# Autodesk Inventor assembly: A-01-0
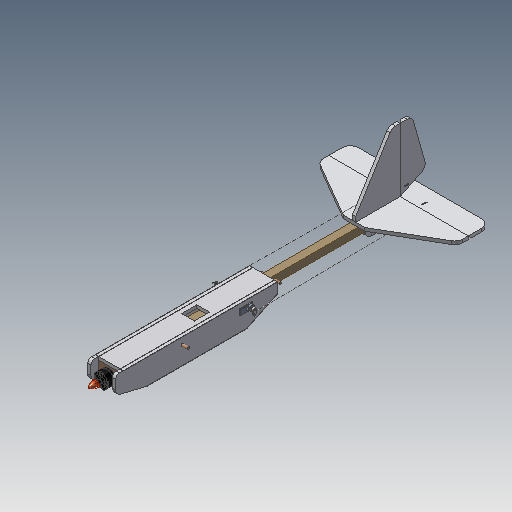
[picture p0: Inventor's stored thumbnail of the model, 512x512]
Saved by Autodesk Inventor 2019 (Build 230136000, 136)
## iProperties
Created: 2022-04-10
Part Number: A-01-0
Document SubType Name: Assembly
Designer: solyo
Mass: 81.7196 g
Surface Area: 1876.72 cm^2
Volume: 370.282 cm^3
Density: 0.220695 g/cm^3
Author: solyo
## Documents named in this file (22)
- D:\Modelling\RC\RC Trainer V1\ASSEMBLY\A-01-0-FUSELAGE\A-01-0.iam
- D:\Modelling\RC\RC Trainer V1\Parts\PW-00-0-TAILBOOM\PW-00-0-0.ipt
- D:\Modelling\RC\RC Trainer V1\Parts\PW-01-0-FIREWALL\PW-01-0-0.ipt
- D:\Modelling\RC\RC Trainer V1\PARTS\PW-02-0-PIN\PW-02-0-0\WING_FRONT_TIE.ipt
- D:\Modelling\RC\RC Trainer V1\Parts\PW-02-0-PIN\PW-02-0-0\WING_REAR_TIE.ipt
- D:\Modelling\RC\RC Trainer V1\Parts\PF-01-0-FUSELAGE\PF-01-0-1.ipt
- D:\Modelling\RC\RC Trainer V1\Parts\C-01-0-EMAX_MT1806_2280KV\C-01-0.ipt
- D:\Modelling\RC\RC Trainer V1\Parts\PF-02-0-HORIZONTAL_STABILIZER\PF-02-0-0.ipt
- D:\Modelling\RC\RC Trainer V1\Parts\PF-03-0-VERTICAL_STABILIZER\PF-03-0-0.ipt
- D:\Modelling\RC\RC Trainer V1\Parts\PW-02-0-PIN\PW-02-0-0\SLIDE.ipt
- D:\Modelling\RC\RC Trainer V1\Parts\PM-00-0-PUSHROD\PM-00-0-0\TAIL.ipt
- D:\Modelling\RC\RC Trainer V1\Parts\PP-00-0-CONTROL_HORN\PP-00-0-0.ipt
- D:\Modelling\RC\RC Trainer V1\Parts\C-02-0-EMAX_12AESC\C-02-0.ipt
- D:\Modelling\RC\RC Trainer V1\Parts\C-03-0-SERVO_3G\C-03-0\CW.ipt
- D:\Modelling\RC\RC Trainer V1\Parts\C-04-0-SERVO_LINKAGE_STOPPER\C-04-0.ipt
- D:\Modelling\RC\RC Trainer V1\Parts\C-05-0-FS2A_4CH\C-05-0.ipt
- D:\Modelling\RC\RC Trainer V1\PARTS\PW-02-0-PIN\PW-02-0-0.ipt
- D:\Modelling\RC\RC Trainer V1\Parts\PM-00-0-PUSHROD\PM-00-0-0.ipt
- D:\Modelling\RC\RC Trainer V1\Parts\C-03-0-SERVO_3G\C-03-0.ipt
- C:\Users\solyo\Documents\Inventor\Content Center Files\R2019\en-US\ISO 7092\ISO 7092 - ST 2 - 140 HV.ipt
- C:\Users\solyo\Documents\Inventor\Content Center Files\R2019\en-US\ISO 4035(2)\ISO 4035 - M2 - ISO.ipt
- C:\Users\solyo\Documents\Inventor\Content Center Files\R2019\en-US\ISO 4762(2)\ISO 4762 - M1.6 x 6ISO.ipt
## Components (25 placed, 18 different names)
1. C-05-0:1 — Mate:39, Mate:40, Mate:41
2. PW-00-0-0:1
3. WING_FRONT_TIE:1
4. WING_REAR_TIE:2
5. ISO 4762 M1.6 x 6:1 — Insert:10
6. ISO 4762 M1.6 x 6:2 — Insert:11
7. C-02-0:1 — Mate:37, Flush:4, Mate:38
8. PW-01-0-0:1 — Flush:4, Mate:38, Mate:41, Mate:44, Mate:45, Mate:46, Insert:10, Insert:11
9. PF-01-0-1:1 — Flush:3, Mate:37, Mate:39, Mate:40
10. C-01-0:1 — Mate:44, Mate:45, Mate:46
11. CW:1
12. CW:2
13. ISO 7092 ST 2 - 140 HV:1 — Insert:6, Insert:8
14. ISO 7092 ST 2 - 140 HV:2 — Insert:7, Insert:9
15. ISO 4035 M2:1 — Insert:8, Mate:49
16. ISO 4035 M2:2 — Insert:9
17. SLIDE:3
18. PF-02-0-0:1 — Mate:14, Mate:43, Mate:48
19. PF-03-0-0:1 — Mate:42
20. TAIL:1
21. TAIL:2
22. PP-00-0-0:1 — Mate:14, Mate:43, Insert:7, Mate:47, Mate:48
23. PP-00-0-0:2 — Mate:42, Insert:6, Mate:50
24. C-04-0:1 — Mate:49, Mate:50
25. C-04-0:2 — Mate:47
## Relationships (55: Mate 43, Insert 8, Flush 4)
- [Mate]: PW-00-0-0:1 ↔ PW-01-0-0:1
- [Flush]: PW-00-0-0:1 ↔ PW-01-0-0:1
- [Mate]: PW-00-0-0:1 ↔ PF-01-0-1:1
- [Mate]: PW-01-0-0:1 ↔ PF-01-0-1:1
- [Mate]: PF-02-0-0:1 ↔ PF-03-0-0:1
- [Mate]: PF-02-0-0:1 ↔ PF-03-0-0:1
- [Mate]: PF-02-0-0:1 ↔ PF-03-0-0:1
- [Mate]: PW-00-0-0:1 ↔ PF-03-0-0:1
- [Mate]: PW-00-0-0:1 ↔ PF-02-0-0:1
- [Mate]: PW-00-0-0:1 ↔ PF-03-0-0:1
- [Mate] (-2.5 mm): SLIDE:3 ↔ PF-03-0-0:1
- [Flush]: SLIDE:3 ↔ PF-03-0-0:1
- Mate:14: PF-02-0-0:1 ↔ PP-00-0-0:1
- [Mate]: PF-03-0-0:1 ↔ PP-00-0-0:2
- [Mate]: PW-00-0-0:1 ↔ CW:1
- [Mate]: PF-01-0-1:1 ↔ CW:1
- [Mate]: PW-00-0-0:1 ↔ CW:2
- [Mate]: PF-01-0-1:1 ↔ CW:2
- [Mate]: PF-01-0-1:1 ↔ CW:2
- [Mate] (10 mm): PF-02-0-0:1 ↔ PP-00-0-0:2
- [Mate]: PF-01-0-1:1 ↔ CW:1
- [Mate]: TAIL:1 ↔ C-04-0:2
- [Mate]: CW:2 ↔ TAIL:1
- [Mate] (1 mm): CW:2 ↔ TAIL:1
- [Insert] (-26 mm): PW-00-0-0:1 ↔ WING_FRONT_TIE:1
- [Mate]: WING_FRONT_TIE:1 ↔ PF-01-0-1:1
- [Insert] (-20 mm): PW-00-0-0:1 ↔ WING_REAR_TIE:2
- [Mate]: SLIDE:3 ↔ PF-03-0-0:1
- [Mate]: CW:1 ↔ TAIL:2
- [Mate] (1 mm): CW:1 ↔ TAIL:2
- [Mate]: TAIL:2 ↔ C-04-0:1
- [Mate]: CW:1 ↔ TAIL:2
- [Mate]: TAIL:2 ↔ C-04-0:1
- Flush:3: PF-01-0-1:1
- Mate:37: C-02-0:1 ↔ PF-01-0-1:1
- Flush:4: C-02-0:1 ↔ PW-01-0-0:1
- Mate:38 (10 mm): C-02-0:1 ↔ PW-01-0-0:1
- Mate:39: C-05-0:1 ↔ PF-01-0-1:1
- Mate:40: C-05-0:1 ↔ PF-01-0-1:1
- Mate:41 (15 mm): C-05-0:1 ↔ PW-01-0-0:1
- Mate:42: PF-03-0-0:1 ↔ PP-00-0-0:2
- Mate:43: PF-02-0-0:1 ↔ PP-00-0-0:1
- Mate:44: PW-01-0-0:1 ↔ C-01-0:1
- Mate:45: PW-01-0-0:1 ↔ C-01-0:1
- Mate:46: PW-01-0-0:1 ↔ C-01-0:1
- Insert:6: ISO 7092 ST 2 - 140 HV:1 ↔ PP-00-0-0:2
- Insert:7: ISO 7092 ST 2 - 140 HV:2 ↔ PP-00-0-0:1
- Insert:8: ISO 7092 ST 2 - 140 HV:1 ↔ ISO 4035 M2:1
- Insert:9: ISO 7092 ST 2 - 140 HV:2 ↔ ISO 4035 M2:2
- Insert:10: ISO 4762 M1.6 x 6:1 ↔ PW-01-0-0:1
- Insert:11: ISO 4762 M1.6 x 6:2 ↔ PW-01-0-0:1
- Mate:47: PP-00-0-0:1 ↔ C-04-0:2
- Mate:48: PF-02-0-0:1 ↔ PP-00-0-0:1
- Mate:49: ISO 4035 M2:1 ↔ C-04-0:1
- Mate:50: PP-00-0-0:2 ↔ C-04-0:1
## Named parameters: d37_d41 = 0 mm
